# Autodesk Inventor assembly: CirculinaNode
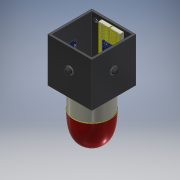
[picture p0: Inventor's stored thumbnail of the model, 180x180]
Saved by Autodesk Inventor 2019 (Build 230136000, 136)
## iProperties
Created: 2019-06-21
Part Number: CirculinaNode
Material: Generic
Document SubType Name: Assembly
Designer: hecto
Author: hecto
## Documents named in this file (10)
- D:\Hackaton\CAD\CirculinaNode.iam
- D:\Hackaton\CAD\Circulina\Circulina.ipt
- D:\Hackaton\CAD\Circulina\Rubber.ipt
- D:\Hackaton\CAD\Case\Case1.ipt
- D:\Hackaton\CAD\Circulina\Sujetador.ipt
- D:\Hackaton\CAD\ContentCenter\en-US\DIN EN ISO 7089\DIN EN ISO 7089 -  3.ipt
- D:\Hackaton\CAD\ContentCenter\en-US\DIN EN ISO 4036\DIN EN ISO 4036 - M3.ipt
- D:\Hackaton\CAD\MQ\MQ_New.ipt
- D:\Hackaton\CAD\ESP32\ESP32S.ipt
- D:\Hackaton\CAD\ESP32\Breadboard2.ipt
## Components (19 placed, 9 different names)
1. Circulina:1 — Flush:1, Flush:2, Mate:1, Mate:2, Mate:3, Mate:4, Mate:5, Mate:6, Mate:7, Mate:8, Mate:9, Mate:12, Mate:14, Mate:16, Mate:18, Mate:20, Mate:22, Mate:24, Mate:26, Mate:28
2. Rubber:1 — Mate:2, Mate:3, Mate:11
3. Rubber:2 — Mate:4, Mate:5, Mate:10, Mate:13
4. Rubber:3 — Mate:6, Mate:7, Mate:15
5. Case1:1 — Mate:8, Mate:9, Mate:10, Mate:29, Mate:30, Angle:1, Mate:31, Mate:32, Mate:33, Angle:2, Mate:34, Angle:3, Mate:39, Flush:41, Mate:40
6. Sujetador:1 — Mate:11, Mate:12, Mate:17
7. Sujetador:2 — Mate:13, Mate:14, Mate:21
8. Sujetador:3 — Mate:15, Mate:16, Mate:19
9. DIN EN ISO 7089 3:1 — Mate:21, Mate:22, Mate:23
10. DIN EN ISO 7089 3:2 — Mate:19, Mate:20, Mate:27
11. DIN EN ISO 7089 3:3 — Mate:17, Mate:18, Mate:25
12. DIN EN ISO 4036 M3:1 — Mate:23, Mate:24
13. DIN EN ISO 4036 M3:2 — Mate:27, Mate:28
14. DIN EN ISO 4036 M3:3 — Mate:25, Mate:26
15. MQ_New:1 — Mate:29, Mate:30, Angle:1
16. MQ_New:2 — Mate:31, Mate:34, Angle:3
17. MQ_New:3 — Mate:32, Mate:33, Angle:2
18. ESP32S:1 — Mate:36, Mate:37, Mate:38
19. Breadboard2:1 — Mate:36, Mate:37, Mate:38, Mate:39, Flush:41, Mate:40
## Relationships (45: Mate 39, Flush 3, Angle 3)
- Flush:1: Circulina:1
- Flush:2: Circulina:1
- Mate:1: Circulina:1
- Mate:2: Circulina:1 ↔ Rubber:1
- Mate:3: Circulina:1 ↔ Rubber:1
- Mate:4: Circulina:1 ↔ Rubber:2
- Mate:5: Circulina:1 ↔ Rubber:2
- Mate:6: Circulina:1 ↔ Rubber:3
- Mate:7: Circulina:1 ↔ Rubber:3
- Mate:8: Circulina:1 ↔ Case1:1
- Mate:9: Circulina:1 ↔ Case1:1
- Mate:10: Rubber:2 ↔ Case1:1
- Mate:11: Rubber:1 ↔ Sujetador:1
- Mate:12: Circulina:1 ↔ Sujetador:1
- Mate:13: Rubber:2 ↔ Sujetador:2
- Mate:14: Circulina:1 ↔ Sujetador:2
- Mate:15: Rubber:3 ↔ Sujetador:3
- Mate:16: Circulina:1 ↔ Sujetador:3
- Mate:17: Sujetador:1 ↔ DIN EN ISO 7089 3:3
- Mate:18: Circulina:1 ↔ DIN EN ISO 7089 3:3
- Mate:19: Sujetador:3 ↔ DIN EN ISO 7089 3:2
- Mate:20: Circulina:1 ↔ DIN EN ISO 7089 3:2
- Mate:21: Sujetador:2 ↔ DIN EN ISO 7089 3:1
- Mate:22: Circulina:1 ↔ DIN EN ISO 7089 3:1
- Mate:23: DIN EN ISO 7089 3:1 ↔ DIN EN ISO 4036 M3:1
- Mate:24: Circulina:1 ↔ DIN EN ISO 4036 M3:1
- Mate:25: DIN EN ISO 7089 3:3 ↔ DIN EN ISO 4036 M3:3
- Mate:26: Circulina:1 ↔ DIN EN ISO 4036 M3:3
- Mate:27: DIN EN ISO 7089 3:2 ↔ DIN EN ISO 4036 M3:2
- Mate:28: Circulina:1 ↔ DIN EN ISO 4036 M3:2
- Mate:29: Case1:1 ↔ MQ_New:1
- Mate:30: Case1:1 ↔ MQ_New:1
- Angle:1 (0 deg): Case1:1 ↔ MQ_New:1
- Mate:31: Case1:1 ↔ MQ_New:2
- Mate:32: Case1:1 ↔ MQ_New:3
- Mate:33: Case1:1 ↔ MQ_New:3
- Angle:2 (0 deg): Case1:1 ↔ MQ_New:3
- Mate:34: Case1:1 ↔ MQ_New:2
- Angle:3 (0 deg): Case1:1 ↔ MQ_New:2
- Mate:36: ESP32S:1 ↔ Breadboard2:1
- Mate:37: ESP32S:1 ↔ Breadboard2:1
- Mate:38: ESP32S:1 ↔ Breadboard2:1
- Mate:39: Case1:1 ↔ Breadboard2:1
- Flush:41 (5 mm): Case1:1 ↔ Breadboard2:1
- Mate:40 (20 mm): Case1:1 ↔ Breadboard2:1
